# Autodesk Inventor assembly: PanelMount
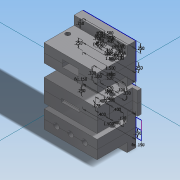
[picture p0: Inventor's stored thumbnail of the model, 180x180]
Saved by Autodesk Inventor 2014 SP2 (Build 180246200, 246)
## iProperties
Created: 2014-06-06
Part Number: PanelMount
Document SubType Name: Assembly
Designer: dliu
Author: dliu
## Documents named in this file (4)
- C:\Users\dliu\Dropbox\dbhome\electric-longboard\dliu\Electronics\PanelMount.iam
- C:\Users\dliu\Dropbox\dbhome\electric-longboard\dliu\Electronics\balance plug holder.ipt
- C:\Users\dliu\Dropbox\dbhome\electric-longboard\dliu\Electronics\keyhole holder.ipt
- C:\Users\dliu\Dropbox\dbhome\electric-longboard\dliu\Electronics\xt-60 holder.ipt
## Components (6 placed, 3 different names)
1. balance plug holder:1 — Mate:1, Mate:4, Mate:7, Mate:8, Flush:2, Flush:5
2. keyhole holder:1 — Mate:2, Mate:5, Mate:7, Flush:3, Flush:4
3. xt-60 holder:1 — Mate:3, Mate:6, Mate:8, Flush:1
4. balance plug holder:3 — Mate:1, Mate:4, Flush:2, Flush:4
5. keyhole holder:3 — Mate:2, Mate:5, Flush:3
6. xt-60 holder:3 — Mate:3, Mate:6, Flush:1, Flush:5
## Relationships (13: Mate 8, Flush 5)
- Mate:1: balance plug holder:1 ↔ balance plug holder:3
- Mate:2: keyhole holder:1 ↔ keyhole holder:3
- Mate:3: xt-60 holder:1 ↔ xt-60 holder:3
- Mate:4: balance plug holder:1 ↔ balance plug holder:3
- Mate:5: keyhole holder:1 ↔ keyhole holder:3
- Mate:6: xt-60 holder:1 ↔ xt-60 holder:3
- Mate:7: balance plug holder:1 ↔ keyhole holder:1
- Mate:8: balance plug holder:1 ↔ xt-60 holder:1
- Flush:1: xt-60 holder:1 ↔ xt-60 holder:3
- Flush:2: balance plug holder:1 ↔ balance plug holder:3
- Flush:3: keyhole holder:1 ↔ keyhole holder:3
- Flush:4: keyhole holder:1 ↔ balance plug holder:3
- Flush:5: balance plug holder:1 ↔ xt-60 holder:3
